# Autodesk Inventor assembly: green-house
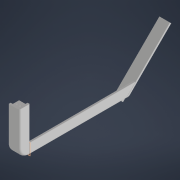
[picture p0: Inventor's stored thumbnail of the model, 180x180]
Saved by Autodesk Inventor 2021 (Build 250183000, 183)
## iProperties
Created: 2020-05-09
Part Number: green-house
Document SubType Name: Assembly
Designer: Jonathan
Author: Jonathan
## Documents named in this file (4)
- C:\Users\Jonathan\green-house\green-house.iam
- C:\Users\Jonathan\green-house\frame.ipt
- C:\Users\Jonathan\green-house\frame-roof.ipt
- C:\Users\Jonathan\green-house\frame-foot.ipt
## Components (3 placed, 3 different names)
1. frame:1 — Rotational:1, Flush:1, Flush:2
2. frame-roof:1 — Rotational:1
3. frame-foot:1 — Flush:1, Flush:2
## Relationships (3: Flush 2, RevoluteJoint 1)
- Rotational:1 [RevoluteJoint]: frame:1 ↔ frame-roof:1
- Flush:1: frame:1 ↔ frame-foot:1
- Flush:2: frame:1 ↔ frame-foot:1
